# Autodesk Inventor assembly: 092_CPY_CPY
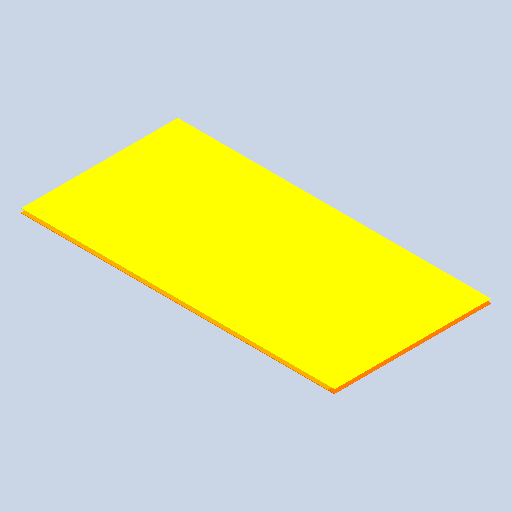
[picture p0: Inventor's stored thumbnail of the model, 512x512]
Saved by Autodesk Inventor 2026 (Build 300175000, 175)
## iProperties
Created: 2026-05-19
Part Number: 092_CPY_CPY
Document SubType Name: Assembly
Designer: user
Author: user
## Documents named in this file (4)
- C:\Users\user\Documents\Inventor\GBK-Gubkinskiy\092_CPY_CPY.iam
- C:\Users\user\Documents\Inventor\GBK-Gubkinskiy\0921_CPY_CPY.ipt
- C:\Users\user\Documents\Inventor\GBK-Gubkinskiy\0922_CPY_CPY.ipt
- C:\Users\user\Documents\Inventor\GBK-Gubkinskiy\0923_CPY_CPY.ipt
## Components (3 placed, 3 different names)
1. 0921_CPY_CPY:1 — Совмещение:1, Заподлицо:1, Заподлицо:2
2. 0922_CPY_CPY:1 — Совмещение:1, Заподлицо:1, Жесткий:1
3. 0923_CPY_CPY:1 — Заподлицо:2, Жесткий:1
## Relationships (4: Flush 2, Mate 1, WeldJoint 1)
- Совмещение:1 [Mate]: 0921_CPY_CPY:1 ↔ 0922_CPY_CPY:1
- Заподлицо:1 [Flush] (34 mm): 0921_CPY_CPY:1 ↔ 0922_CPY_CPY:1
- Заподлицо:2 [Flush] (34 mm): 0921_CPY_CPY:1 ↔ 0923_CPY_CPY:1
- Жесткий:1 [WeldJoint]: 0922_CPY_CPY:1 ↔ 0923_CPY_CPY:1
